# Autodesk Inventor assembly: holder_to_grab
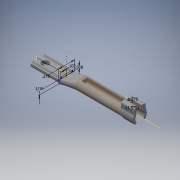
[picture p0: Inventor's stored thumbnail of the model, 180x180]
Saved by Autodesk Inventor 2016 (Build 200138000, 138)
## iProperties
Created: 2016-09-02
Part Number: holder_to_grab
Document SubType Name: Assembly
Designer: GentnerLab
Author: GentnerLab
## Documents named in this file (3)
- C:\Users\GentnerLab\Documents\Inventor\Parts\new_drive\holder_to_grab.iam
- C:\Users\GentnerLab\Documents\Inventor\Parts\new_drive\60unm-6mm\derived_drive_holder.ipt
- C:\Users\GentnerLab\Documents\GentnerLabSTL\2-reel_holder.ipt
## Components (2 placed, 2 different names)
1. derived_drive_holder:1 — Mate:1, Mate:2
2. 2-reel_holder:1 — Mate:1, Mate:2
## Relationships (2: Mate 2)
- Mate:1: derived_drive_holder:1 ↔ 2-reel_holder:1
- Mate:2: derived_drive_holder:1 ↔ 2-reel_holder:1
